# Autodesk Inventor assembly: Aufbau1,0
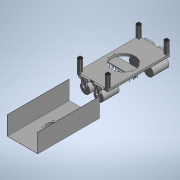
[picture p0: Inventor's stored thumbnail of the model, 180x180]
Saved by Autodesk Inventor 2021.3 (Build 253353000, 353)
## iProperties
Created: 2021-10-11
Part Number: Aufbau1,0
Document SubType Name: Baugruppe
Designer: bhelg
Author: bhelg
## Documents named in this file (10)
- P:\Benutzer\bhelg\Inventor\Christoph Bärtschi\Gruppe Wennemers\Jonas Rackl UV Box\Aufbau1,0.iam
- P:\Benutzer\bhelg\Inventor\Christoph Bärtschi\Gruppe Wennemers\Jonas Rackl UV Box\Grundplatte1.0.ipt
- P:\Benutzer\bhelg\Inventor\Christoph Bärtschi\Gruppe Wennemers\Jonas Rackl UV Box\Lampenhalterung1,0.ipt
- P:\Benutzer\bhelg\Inventor\Christoph Bärtschi\Gruppe Wennemers\Jonas Rackl UV Box\20x20Profil 1.0.ipt
- P:\Benutzer\bhelg\Inventor\Christoph Bärtschi\Gruppe Wennemers\Jonas Rackl UV Box\Wobatech Abdeckkappe 20x20.ipt
- P:\Benutzer\bhelg\Inventor\Christoph Bärtschi\Gruppe Wennemers\Jonas Rackl UV Box\Lampe.ipt
- P:\Benutzer\bhelg\Inventor\Christoph Bärtschi\Gruppe Wennemers\Jonas Rackl UV Box\Deckel1,0.ipt
- P:\Benutzer\bhelg\Inventor\Christoph Bärtschi\Gruppe Wennemers\Jonas Rackl UV Box\Lüfter80x80.ipt
- P:\Benutzer\bhelg\Inventor\Christoph Bärtschi\Gruppe Wennemers\Jonas Rackl UV Box\Halterung Gläser1,0.ipt
- P:\Benutzer\bhelg\Inventor\Christoph Bärtschi\Gruppe Wennemers\Jonas Rackl UV Box\Glas klein.ipt
## Components (21 placed, 9 different names)
1. Grundplatte1.0:1 — Fluchtend:1, Fluchtend:2, Fluchtend:3, Passend:1, Winkel:1, Tangential:1, Passend:2, Passend:3, Passend:4, Einfügen:1, Einfügen:2, Einfügen:3, Einfügen:4, Passend:5, Passend:6, Passend:8, Winkel:3, Einfügen:15
2. Lampenhalterung1,0:1 — Passend:1, Winkel:1, Tangential:1, Fluchtend:4, Fluchtend:5, Fluchtend:6, Einfügen:10
3. Lampenhalterung1,0:2 — Fluchtend:5, Passend:4, Einfügen:12
4. Lampenhalterung1,0:3 — Fluchtend:6, Passend:3, Einfügen:13
5. Lampenhalterung1,0:4 — Passend:2, Fluchtend:4, Einfügen:9
6. 20x20Profil 1.0:1 — Einfügen:1, Einfügen:7
7. 20x20Profil 1.0:2 — Einfügen:2, Einfügen:8
8. 20x20Profil 1.0:3 — Einfügen:3, Einfügen:6
9. 20x20Profil 1.0:4 — Einfügen:4, Einfügen:5
10. Wobatech Abdeckkappe 20x20:1 — Einfügen:6
11. Wobatech Abdeckkappe 20x20:2 — Einfügen:5
12. Wobatech Abdeckkappe 20x20:3 — Einfügen:7
13. Wobatech Abdeckkappe 20x20:4 — Einfügen:8
14. Lampe:1 — Einfügen:9
15. Lampe:2 — Einfügen:12
16. Lampe:3 — Einfügen:13
17. Lampe:4 — Einfügen:10
18. Deckel1,0:1 — Passend:5, Passend:6, Passend:7, Winkel:2, Einfügen:14
19. Lüfter80x80:1 — Passend:7, Winkel:2, Einfügen:14
20. Halterung Gläser1,0:1 — Passend:8, Winkel:3, Einfügen:15, Passend:9
21. Glas klein:1 — Passend:9
## Relationships (33: Insert 14, Mate 9, Flush 6, Angle 3, Tangent 1)
- Fluchtend:1 [Flush]: Grundplatte1.0:1
- Fluchtend:2 [Flush]: Grundplatte1.0:1
- Fluchtend:3 [Flush]: Grundplatte1.0:1
- Passend:1 [Mate]: Grundplatte1.0:1 ↔ Lampenhalterung1,0:1
- Winkel:1 [Angle] (0 deg): Grundplatte1.0:1 ↔ Lampenhalterung1,0:1
- Tangential:1 (0.483 mm): Grundplatte1.0:1 ↔ Lampenhalterung1,0:1
- Passend:2 [Mate]: Grundplatte1.0:1 ↔ Lampenhalterung1,0:4
- Fluchtend:4 [Flush]: Lampenhalterung1,0:1 ↔ Lampenhalterung1,0:4
- Fluchtend:5 [Flush]: Lampenhalterung1,0:1 ↔ Lampenhalterung1,0:2
- Fluchtend:6 [Flush]: Lampenhalterung1,0:1 ↔ Lampenhalterung1,0:3
- Passend:3 [Mate]: Grundplatte1.0:1 ↔ Lampenhalterung1,0:3
- Passend:4 [Mate]: Grundplatte1.0:1 ↔ Lampenhalterung1,0:2
- Einfügen:1 [Insert]: Grundplatte1.0:1 ↔ 20x20Profil 1.0:1
- Einfügen:2 [Insert]: Grundplatte1.0:1 ↔ 20x20Profil 1.0:2
- Einfügen:3 [Insert]: Grundplatte1.0:1 ↔ 20x20Profil 1.0:3
- Einfügen:4 [Insert]: Grundplatte1.0:1 ↔ 20x20Profil 1.0:4
- Einfügen:5 [Insert] (-7 mm): 20x20Profil 1.0:4 ↔ Wobatech Abdeckkappe 20x20:2
- Einfügen:6 [Insert] (-7 mm): 20x20Profil 1.0:3 ↔ Wobatech Abdeckkappe 20x20:1
- Einfügen:7 [Insert] (-7 mm): 20x20Profil 1.0:1 ↔ Wobatech Abdeckkappe 20x20:3
- Einfügen:8 [Insert] (-7 mm): 20x20Profil 1.0:2 ↔ Wobatech Abdeckkappe 20x20:4
- Einfügen:9 [Insert]: Lampenhalterung1,0:4 ↔ Lampe:1
- Einfügen:10 [Insert]: Lampenhalterung1,0:1 ↔ Lampe:4
- Einfügen:12 [Insert]: Lampenhalterung1,0:2 ↔ Lampe:2
- Einfügen:13 [Insert]: Lampenhalterung1,0:3 ↔ Lampe:3
- Passend:5 [Mate]: Grundplatte1.0:1 ↔ Deckel1,0:1
- Passend:6 [Mate]: Grundplatte1.0:1 ↔ Deckel1,0:1
- Passend:7 [Mate]: Deckel1,0:1 ↔ Lüfter80x80:1
- Winkel:2 [Angle] (0 deg): Deckel1,0:1 ↔ Lüfter80x80:1
- Einfügen:14 [Insert]: Deckel1,0:1 ↔ Lüfter80x80:1
- Passend:8 [Mate]: Grundplatte1.0:1 ↔ Halterung Gläser1,0:1
- Winkel:3 [Angle] (0 deg): Grundplatte1.0:1 ↔ Halterung Gläser1,0:1
- Einfügen:15 [Insert]: Grundplatte1.0:1 ↔ Halterung Gläser1,0:1
- Passend:9 [Mate]: Halterung Gläser1,0:1 ↔ Glas klein:1
